# Autodesk Inventor assembly: EL2-400A
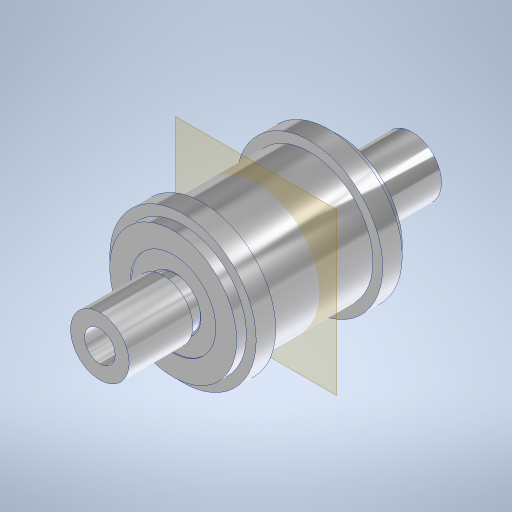
[picture p0: Inventor's stored thumbnail of the model, 512x512]
Saved by Autodesk Inventor 2023.4 (Build 274418000, 418)
## iProperties
Created: 2025-01-11
Part Number: EL2-400A
Document SubType Name: Assembly
Designer: mavericks
Author: mavericks
## Documents named in this file (4)
- C:\Users\mavericks\Documents\Robotics\GitHub\2025-ReefScape---CAD\Elevator\EL2\EL2-400A.iam
- C:\Users\mavericks\Documents\Robotics\GitHub\2025-ReefScape---CAD\Elevator\EL2\EL2-007.ipt
- C:\Users\mavericks\Documents\Robotics\GitHub\2025-ReefScape---CAD\Elevator\EL2\EL2-008.ipt
- C:\Users\mavericks\Documents\Robotics\GitHub\2025-ReefScape---CAD\COMMON PARTS\BEARINGS\.25_Bearing_ext_race.ipt
## Components (5 placed, 3 different names)
1. EL2-007:1 — Mate:1, Mate:2, Mate:3, Mate:4
2. EL2-008:1 — Mate:5, Mate:6
3. EL2-008:2 — Mate:7, Mate:8
4. .25_Bearing_ext_race:1 — Mate:3, Mate:4, Mate:5, Mate:6
5. .25_Bearing_ext_race:2 — Mate:1, Mate:2, Mate:7, Mate:8
## Relationships (8: Mate 8)
- Mate:1: EL2-007:1 ↔ .25_Bearing_ext_race:2
- Mate:2: EL2-007:1 ↔ .25_Bearing_ext_race:2
- Mate:3: EL2-007:1 ↔ .25_Bearing_ext_race:1
- Mate:4: EL2-007:1 ↔ .25_Bearing_ext_race:1
- Mate:5: EL2-008:1 ↔ .25_Bearing_ext_race:1
- Mate:6: EL2-008:1 ↔ .25_Bearing_ext_race:1
- Mate:7: EL2-008:2 ↔ .25_Bearing_ext_race:2
- Mate:8: EL2-008:2 ↔ .25_Bearing_ext_race:2
